# Autodesk Inventor assembly: Board Assembly
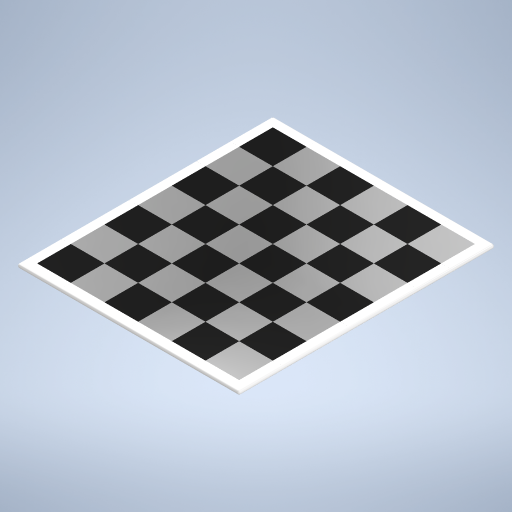
[picture p0: Inventor's stored thumbnail of the model, 512x512]
Saved by Autodesk Inventor 2023.1 (Build 271208000, 208)
## iProperties
Created: 2023-04-17
Part Number: Board Assembly
Document SubType Name: Assembly
Designer: czha626
Author: czha626
## Documents named in this file (9)
- C:\Users\czha626\OneDrive - The University of Auckland\Publications\Paper 2\Figures\Calibration target\Board Assembly.iam
- C:\Users\czha626\OneDrive - The University of Auckland\Publications\Paper 2\Calibration board\Calibration board\BoardNew2-CZ.ipt
- C:\Users\czha626\OneDrive - The University of Auckland\Publications\Paper 2\Calibration board\Calibration board\Connecter-CZ.ipt
- C:\Users\czha626\OneDrive - The University of Auckland\Publications\Paper 2\Calibration board\Calibration board\Boardborder.ipt
- C:\Users\czha626\OneDrive - The University of Auckland\Publications\Paper 2\Calibration board\Calibration board\Boardborder1.ipt
- C:\Users\czha626\OneDrive - The University of Auckland\Publications\Paper 2\Calibration board\Calibration board\Boardborder4.ipt
- C:\Users\czha626\OneDrive - The University of Auckland\Publications\Paper 2\Calibration board\Calibration board\Boardborder3.ipt
- C:\Users\czha626\OneDrive - The University of Auckland\Publications\Paper 2\Calibration board\Calibration board\Boardborder2.ipt
- C:\Users\czha626\OneDrive - The University of Auckland\Publications\Paper 2\Figures\Calibration target\Aluminium.ipt
## Components (132 placed, 8 different names)
1. BoardNew2-CZ:1 — Mate:1, Flush:1, Mate:2, Mate:3, Mate:4, Mate:5, Mate:7, Flush:2, Mate:29, Flush:9, Flush:10, Mate:31, Mate:32, Mate:34, Mate:52, Mate:53, Mate:54, Mate:198, Mate:199, Mate:209, Mate:259, Flush:46, Mate:326, Mate:328, Mate:329
2. Connecter-CZ:1 — Mate:19, Mate:20, Mate:21
3. Connecter-CZ:2 — Mate:16, Mate:17, Mate:18
4. Connecter-CZ:3 — Mate:2, Mate:3, Mate:4
5. Connecter-CZ:4 — Mate:5, Mate:6, Mate:7
6. BoardNew2-CZ:2 — Mate:1, Flush:1, Mate:6, Flush:2, Mate:15, Flush:5, Flush:6, Mate:16, Mate:21, Mate:49, Mate:50, Mate:51, Mate:196, Mate:197, Mate:210, Mate:311, Mate:320, Mate:325
7. BoardNew2-CZ:3 — Mate:15, Flush:5, Flush:6, Mate:17, Mate:18, Mate:19, Mate:20, Mate:46, Mate:47, Mate:48, Mate:194, Mate:195, Mate:211, Mate:257, Flush:45, Mate:319
8. Connecter-CZ:5
9. Connecter-CZ:6
10. BoardNew2-CZ:4 — Mate:43, Mate:44, Mate:45, Mate:127, Flush:25, Flush:26, Mate:192, Mate:193, Mate:212, Mate:213, Mate:214, Mate:215, Mate:216, Mate:217, Mate:230, Mate:255, Mate:256, Flush:44, Flush:54, Mate:322
11. BoardNew2-CZ:5 — Flush:11, Flush:12, Mate:36, Mate:37, Mate:39, Mate:40, Mate:42, Mate:58, Mate:59, Mate:60, Mate:202, Mate:203, Mate:207, Mate:265, Flush:49, Mate:332, Mate:334
12. Connecter-CZ:9
13. Connecter-CZ:10
14. BoardNew2-CZ:6 — Mate:29, Flush:9, Flush:10, Mate:30, Mate:33, Mate:35, Mate:55, Mate:56, Mate:57, Mate:200, Mate:201, Mate:208, Mate:330, Mate:331, Mate:333
15. Connecter-CZ:11 — Mate:192, Mate:193, Mate:212
16. Connecter-CZ:12 — Mate:30, Mate:31, Mate:32
17. Connecter-CZ:13 — Mate:33, Mate:34, Mate:35
18. BoardNew2-CZ:7 — Flush:11, Flush:12, Mate:36, Mate:38, Mate:41, Mate:61, Mate:62, Mate:63, Mate:204, Mate:205, Mate:206, Mate:231, Mate:232, Mate:233, Mate:234, Mate:243, Mate:244, Mate:249, Mate:250, Flush:41, Flush:51, Mate:302, Mate:335, Mate:337, Mate:339
19. Connecter-CZ:14 — Mate:40, Mate:41, Mate:42
20. Connecter-CZ:15 — Mate:37, Mate:38, Mate:39
21. Connecter-CZ:16 — Mate:43, Mate:44, Mate:45
22. Connecter-CZ:17 — Mate:49, Mate:50, Mate:51
23. Connecter-CZ:18 — Mate:52, Mate:53, Mate:54
24. Connecter-CZ:19 — Mate:46, Mate:47, Mate:48
25. Connecter-CZ:20 — Mate:55, Mate:56, Mate:57
26. Connecter-CZ:21 — Mate:58, Mate:59, Mate:60
27. Connecter-CZ:22 — Mate:61, Mate:62, Mate:63
28. BoardNew2-CZ:8 — Mate:305, Mate:307, Mate:312
29. Connecter-CZ:23
30. Connecter-CZ:24
31. Connecter-CZ:25
32. Connecter-CZ:26
33. BoardNew2-CZ:9 — Mate:285, Mate:310, Mate:315
34. BoardNew2-CZ:10 — Mate:313, Mate:314, Mate:317, Mate:321
35. Connecter-CZ:27
36. Connecter-CZ:28
37. BoardNew2-CZ:11 — Mate:127, Flush:25, Flush:26, Mate:191, Flush:39, Flush:40, Mate:218, Mate:219, Mate:220, Mate:221, Mate:228, Mate:229, Flush:53, Mate:275, Mate:282, Mate:316, Mate:318
38. BoardNew2-CZ:12 — Mate:298, Mate:336
39. Connecter-CZ:29
40. Connecter-CZ:30
41. BoardNew2-CZ:13 — Mate:291, Mate:300, Mate:304, Mate:306, Mate:309
42. Connecter-CZ:31
43. Connecter-CZ:32
44. BoardNew2-CZ:14 — Mate:235, Mate:236, Mate:237, Mate:238, Mate:245, Mate:246, Flush:52, Mate:301
45. Connecter-CZ:33
46. Connecter-CZ:34
47. Connecter-CZ:35
48. Connecter-CZ:36
49. Connecter-CZ:37
50. Connecter-CZ:38
51. Connecter-CZ:39
52. Connecter-CZ:40
53. Connecter-CZ:41
54. BoardNew2-CZ:15 — Mate:263, Flush:48, Mate:286, Mate:287, Mate:290, Mate:308
55. Connecter-CZ:42
56. Connecter-CZ:43
57. Connecter-CZ:44
58. Connecter-CZ:45
59. BoardNew2-CZ:16 — Mate:278, Mate:283
60. BoardNew2-CZ:17 — Mate:261, Flush:47, Mate:277, Mate:279, Mate:284
61. Connecter-CZ:46
62. Connecter-CZ:47
63. BoardNew2-CZ:18 — Mate:191, Flush:39, Flush:40, Mate:222, Mate:223, Mate:224, Mate:225, Mate:226, Mate:227, Mate:251, Mate:252, Flush:42, Mate:273, Mate:280
64. BoardNew2-CZ:19 — Mate:267, Flush:50, Mate:292, Mate:296, Mate:299
65. Connecter-CZ:48
66. Connecter-CZ:49
67. BoardNew2-CZ:20 — Mate:288, Mate:289, Mate:293
68. Connecter-CZ:50
69. Connecter-CZ:51
70. BoardNew2-CZ:21 — Mate:239, Mate:240, Mate:241, Mate:242, Mate:247, Mate:248, Mate:253, Mate:254, Flush:43, Mate:269, Mate:271, Mate:295, Mate:297
71. Connecter-CZ:52
72. Connecter-CZ:53
73. Connecter-CZ:54
74. Connecter-CZ:55
75. Connecter-CZ:56
76. Connecter-CZ:57
77. Connecter-CZ:58
78. Connecter-CZ:59
79. Connecter-CZ:60
80. Connecter-CZ:61 — Mate:198, Mate:199, Mate:209
81. Connecter-CZ:62 — Mate:200, Mate:201, Mate:208
82. Connecter-CZ:63 — Mate:194, Mate:195, Mate:211
83. Connecter-CZ:64 — Mate:202, Mate:203, Mate:207
84. Connecter-CZ:65 — Mate:204, Mate:205, Mate:206
85. Connecter-CZ:66 — Mate:196, Mate:197, Mate:210
86. Connecter-CZ:67 — Mate:213, Mate:214, Mate:215
87. Connecter-CZ:68 — Mate:216, Mate:217, Mate:230
88. Connecter-CZ:69 — Mate:218, Mate:219, Mate:229
89. Connecter-CZ:70 — Mate:220, Mate:221, Mate:228
90. Connecter-CZ:71 — Mate:222, Mate:223, Mate:227
91. Connecter-CZ:72 — Mate:224, Mate:225, Mate:226
92. Connecter-CZ:73 — Mate:231, Mate:232, Mate:243
93. Connecter-CZ:74 — Mate:233, Mate:234, Mate:244
94. Connecter-CZ:75 — Mate:235, Mate:236, Mate:245
95. Connecter-CZ:76 — Mate:237, Mate:238, Mate:246
96. Connecter-CZ:77 — Mate:239, Mate:240, Mate:247
97. Connecter-CZ:78 — Mate:241, Mate:242, Mate:248
98. Boardborder:1 — Mate:249, Mate:250, Flush:41, Mate:270, Mate:338
99. Boardborder:2 — Mate:251, Mate:252, Flush:42, Mate:262, Mate:274
100. Boardborder1:1 — Mate:253, Mate:254, Flush:43, Mate:268
101. Boardborder1:2 — Mate:255, Mate:256, Flush:44, Mate:258, Mate:276, Mate:323, Mate:324
102. Boardborder4:1 — Mate:257, Mate:258, Flush:45, Mate:260, Mate:327
103. Boardborder4:2 — Mate:261, Flush:47, Mate:262, Mate:264
104. Boardborder4:3 — Mate:259, Flush:46, Mate:260, Mate:266
105. Boardborder4:4 — Mate:263, Flush:48, Mate:264
106. Boardborder3:1 — Mate:267, Mate:268, Flush:50, Mate:294
107. Boardborder3:2 — Mate:265, Flush:49, Mate:266
108. Boardborder2:1 — Mate:269, Mate:270, Flush:51, Mate:272, Mate:303
109. Boardborder2:2 — Mate:271, Mate:272, Flush:52
110. Boardborder2:3 — Mate:275, Mate:276, Flush:54
111. Boardborder2:4 — Mate:273, Mate:274, Flush:53, Mate:281
112. Aluminium:1 — Mate:277, Mate:278, Mate:279
113. Aluminium:2 — Mate:283, Mate:284, Mate:285
114. Aluminium:3 — Mate:280, Mate:281, Mate:282
115. Aluminium:4 — Mate:286, Mate:287, Mate:288
116. Aluminium:5 — Mate:289, Mate:290, Mate:291
117. Aluminium:6 — Mate:292, Mate:293, Mate:294
118. Aluminium:7 — Mate:301, Mate:302, Mate:303
119. Aluminium:8 — Mate:298, Mate:299, Mate:300
120. Aluminium:9 — Mate:295, Mate:296, Mate:297
121. Aluminium:10 — Mate:322, Mate:323, Mate:324
122. Aluminium:11 — Mate:319, Mate:320, Mate:321
123. Aluminium:12 — Mate:310, Mate:311, Mate:312
124. Aluminium:13 — Mate:313, Mate:314, Mate:315
125. Aluminium:14 — Mate:307, Mate:308, Mate:309
126. Aluminium:15 — Mate:304, Mate:305, Mate:306
127. Aluminium:16 — Mate:316, Mate:317, Mate:318
128. Aluminium:17 — Mate:325, Mate:326, Mate:327
129. Aluminium:18 — Mate:337, Mate:338, Mate:339
130. Aluminium:19 — Mate:334, Mate:335, Mate:336
131. Aluminium:20 — Mate:331, Mate:332, Mate:333
132. Aluminium:21 — Mate:328, Mate:329, Mate:330
## Relationships (393: Mate 339, Flush 54)
- Mate:1: BoardNew2-CZ:1 ↔ BoardNew2-CZ:2
- Flush:1: BoardNew2-CZ:1 ↔ BoardNew2-CZ:2
- Mate:2: BoardNew2-CZ:1 ↔ Connecter-CZ:3
- Mate:3: BoardNew2-CZ:1 ↔ Connecter-CZ:3
- Mate:4: BoardNew2-CZ:1 ↔ Connecter-CZ:3
- Mate:5: BoardNew2-CZ:1 ↔ Connecter-CZ:4
- Mate:6: Connecter-CZ:4 ↔ BoardNew2-CZ:2
- Mate:7: BoardNew2-CZ:1 ↔ Connecter-CZ:4
- Flush:2: BoardNew2-CZ:1 ↔ BoardNew2-CZ:2
- [Mate]: BoardNew2-CZ:3 ↔ BoardNew2-CZ:4
- [Flush]: BoardNew2-CZ:3 ↔ BoardNew2-CZ:4
- [Mate]: BoardNew2-CZ:3 ↔ Connecter-CZ:5
- [Mate]: BoardNew2-CZ:3 ↔ Connecter-CZ:5
- [Mate]: BoardNew2-CZ:3 ↔ Connecter-CZ:5
- [Mate]: BoardNew2-CZ:3 ↔ Connecter-CZ:6
- [Mate]: Connecter-CZ:6 ↔ BoardNew2-CZ:4
- [Mate]: BoardNew2-CZ:3 ↔ Connecter-CZ:6
- [Flush]: BoardNew2-CZ:3 ↔ BoardNew2-CZ:4
- Mate:15: BoardNew2-CZ:2 ↔ BoardNew2-CZ:3
- Flush:5: BoardNew2-CZ:2 ↔ BoardNew2-CZ:3
- Flush:6: BoardNew2-CZ:2 ↔ BoardNew2-CZ:3
- Mate:16: Connecter-CZ:2 ↔ BoardNew2-CZ:2
- Mate:17: Connecter-CZ:2 ↔ BoardNew2-CZ:3
- Mate:18: Connecter-CZ:2 ↔ BoardNew2-CZ:3
- Mate:19: Connecter-CZ:1 ↔ BoardNew2-CZ:3
- Mate:20: Connecter-CZ:1 ↔ BoardNew2-CZ:3
- Mate:21: Connecter-CZ:1 ↔ BoardNew2-CZ:2
- [Mate]: BoardNew2-CZ:5 ↔ BoardNew2-CZ:6
- [Flush]: BoardNew2-CZ:5 ↔ BoardNew2-CZ:6
- [Mate]: BoardNew2-CZ:5 ↔ Connecter-CZ:9
- [Mate]: BoardNew2-CZ:5 ↔ Connecter-CZ:9
- [Mate]: BoardNew2-CZ:5 ↔ Connecter-CZ:9
- [Mate]: BoardNew2-CZ:5 ↔ Connecter-CZ:10
- [Mate]: Connecter-CZ:10 ↔ BoardNew2-CZ:6
- [Mate]: BoardNew2-CZ:5 ↔ Connecter-CZ:10
- [Flush]: BoardNew2-CZ:5 ↔ BoardNew2-CZ:6
- Mate:29: BoardNew2-CZ:1 ↔ BoardNew2-CZ:6
- Flush:9: BoardNew2-CZ:1 ↔ BoardNew2-CZ:6
- Flush:10: BoardNew2-CZ:1 ↔ BoardNew2-CZ:6
- Mate:30: BoardNew2-CZ:6 ↔ Connecter-CZ:12
- Mate:31: BoardNew2-CZ:1 ↔ Connecter-CZ:12
- Mate:32: BoardNew2-CZ:1 ↔ Connecter-CZ:12
- Mate:33: BoardNew2-CZ:6 ↔ Connecter-CZ:13
- Mate:34: BoardNew2-CZ:1 ↔ Connecter-CZ:13
- Mate:35: BoardNew2-CZ:6 ↔ Connecter-CZ:13
- Flush:11: BoardNew2-CZ:5 ↔ BoardNew2-CZ:7
- Flush:12: BoardNew2-CZ:5 ↔ BoardNew2-CZ:7
- Mate:36: BoardNew2-CZ:5 ↔ BoardNew2-CZ:7
- Mate:37: BoardNew2-CZ:5 ↔ Connecter-CZ:15
- Mate:38: BoardNew2-CZ:7 ↔ Connecter-CZ:15
- Mate:39: BoardNew2-CZ:5 ↔ Connecter-CZ:15
- Mate:40: BoardNew2-CZ:5 ↔ Connecter-CZ:14
- Mate:41: BoardNew2-CZ:7 ↔ Connecter-CZ:14
- Mate:42: BoardNew2-CZ:5 ↔ Connecter-CZ:14
- Mate:43: BoardNew2-CZ:4 ↔ Connecter-CZ:16
- Mate:44: BoardNew2-CZ:4 ↔ Connecter-CZ:16
- Mate:45: BoardNew2-CZ:4 ↔ Connecter-CZ:16
- Mate:46: BoardNew2-CZ:3 ↔ Connecter-CZ:19
- Mate:47: BoardNew2-CZ:3 ↔ Connecter-CZ:19
- Mate:48: BoardNew2-CZ:3 ↔ Connecter-CZ:19
- Mate:49: BoardNew2-CZ:2 ↔ Connecter-CZ:17
- Mate:50: BoardNew2-CZ:2 ↔ Connecter-CZ:17
- Mate:51: BoardNew2-CZ:2 ↔ Connecter-CZ:17
- Mate:52: BoardNew2-CZ:1 ↔ Connecter-CZ:18
- Mate:53: BoardNew2-CZ:1 ↔ Connecter-CZ:18
- Mate:54: BoardNew2-CZ:1 ↔ Connecter-CZ:18
- Mate:55: BoardNew2-CZ:6 ↔ Connecter-CZ:20
- Mate:56: BoardNew2-CZ:6 ↔ Connecter-CZ:20
- Mate:57: BoardNew2-CZ:6 ↔ Connecter-CZ:20
- Mate:58: BoardNew2-CZ:5 ↔ Connecter-CZ:21
- Mate:59: BoardNew2-CZ:5 ↔ Connecter-CZ:21
- Mate:60: BoardNew2-CZ:5 ↔ Connecter-CZ:21
- Mate:61: BoardNew2-CZ:7 ↔ Connecter-CZ:22
- Mate:62: BoardNew2-CZ:7 ↔ Connecter-CZ:22
- Mate:63: BoardNew2-CZ:7 ↔ Connecter-CZ:22
- [Mate]: BoardNew2-CZ:8 ↔ BoardNew2-CZ:9
- [Flush]: BoardNew2-CZ:8 ↔ BoardNew2-CZ:9
- [Mate]: BoardNew2-CZ:8 ↔ Connecter-CZ:25
- [Mate]: BoardNew2-CZ:8 ↔ Connecter-CZ:25
- [Mate]: BoardNew2-CZ:8 ↔ Connecter-CZ:25
- [Mate]: BoardNew2-CZ:8 ↔ Connecter-CZ:26
- [Mate]: Connecter-CZ:26 ↔ BoardNew2-CZ:9
- [Mate]: BoardNew2-CZ:8 ↔ Connecter-CZ:26
- [Flush]: BoardNew2-CZ:8 ↔ BoardNew2-CZ:9
- [Mate]: BoardNew2-CZ:10 ↔ BoardNew2-CZ:11
- [Flush]: BoardNew2-CZ:10 ↔ BoardNew2-CZ:11
- [Mate]: BoardNew2-CZ:10 ↔ Connecter-CZ:27
- [Mate]: BoardNew2-CZ:10 ↔ Connecter-CZ:27
- [Mate]: BoardNew2-CZ:10 ↔ Connecter-CZ:27
- [Mate]: BoardNew2-CZ:10 ↔ Connecter-CZ:28
- [Mate]: Connecter-CZ:28 ↔ BoardNew2-CZ:11
- [Mate]: BoardNew2-CZ:10 ↔ Connecter-CZ:28
- [Flush]: BoardNew2-CZ:10 ↔ BoardNew2-CZ:11
- [Mate]: BoardNew2-CZ:9 ↔ BoardNew2-CZ:10
- [Flush]: BoardNew2-CZ:9 ↔ BoardNew2-CZ:10
- [Flush]: BoardNew2-CZ:9 ↔ BoardNew2-CZ:10
- [Mate]: Connecter-CZ:24 ↔ BoardNew2-CZ:9
- [Mate]: Connecter-CZ:24 ↔ BoardNew2-CZ:10
- [Mate]: Connecter-CZ:24 ↔ BoardNew2-CZ:10
- [Mate]: Connecter-CZ:23 ↔ BoardNew2-CZ:10
- [Mate]: Connecter-CZ:23 ↔ BoardNew2-CZ:10
- [Mate]: Connecter-CZ:23 ↔ BoardNew2-CZ:9
- [Mate]: BoardNew2-CZ:12 ↔ BoardNew2-CZ:13
- [Flush]: BoardNew2-CZ:12 ↔ BoardNew2-CZ:13
- [Mate]: BoardNew2-CZ:12 ↔ Connecter-CZ:29
- [Mate]: BoardNew2-CZ:12 ↔ Connecter-CZ:29
- [Mate]: BoardNew2-CZ:12 ↔ Connecter-CZ:29
- [Mate]: BoardNew2-CZ:12 ↔ Connecter-CZ:30
- [Mate]: Connecter-CZ:30 ↔ BoardNew2-CZ:13
- [Mate]: BoardNew2-CZ:12 ↔ Connecter-CZ:30
- [Flush]: BoardNew2-CZ:12 ↔ BoardNew2-CZ:13
- [Mate]: BoardNew2-CZ:8 ↔ BoardNew2-CZ:13
- [Flush]: BoardNew2-CZ:8 ↔ BoardNew2-CZ:13
- [Flush]: BoardNew2-CZ:8 ↔ BoardNew2-CZ:13
- [Mate]: BoardNew2-CZ:13 ↔ Connecter-CZ:31
- [Mate]: BoardNew2-CZ:8 ↔ Connecter-CZ:31
- [Mate]: BoardNew2-CZ:8 ↔ Connecter-CZ:31
- [Mate]: BoardNew2-CZ:13 ↔ Connecter-CZ:32
- [Mate]: BoardNew2-CZ:8 ↔ Connecter-CZ:32
- [Mate]: BoardNew2-CZ:13 ↔ Connecter-CZ:32
- [Flush]: BoardNew2-CZ:12 ↔ BoardNew2-CZ:14
- [Flush]: BoardNew2-CZ:12 ↔ BoardNew2-CZ:14
- [Mate]: BoardNew2-CZ:12 ↔ BoardNew2-CZ:14
- [Mate]: BoardNew2-CZ:12 ↔ Connecter-CZ:34
- [Mate]: BoardNew2-CZ:14 ↔ Connecter-CZ:34
- [Mate]: BoardNew2-CZ:12 ↔ Connecter-CZ:34
- [Mate]: BoardNew2-CZ:12 ↔ Connecter-CZ:33
- [Mate]: BoardNew2-CZ:14 ↔ Connecter-CZ:33
- [Mate]: BoardNew2-CZ:12 ↔ Connecter-CZ:33
- [Mate]: BoardNew2-CZ:11 ↔ Connecter-CZ:35
- [Mate]: BoardNew2-CZ:11 ↔ Connecter-CZ:35
- [Mate]: BoardNew2-CZ:11 ↔ Connecter-CZ:35
- [Mate]: BoardNew2-CZ:10 ↔ Connecter-CZ:38
- [Mate]: BoardNew2-CZ:10 ↔ Connecter-CZ:38
- [Mate]: BoardNew2-CZ:10 ↔ Connecter-CZ:38
- [Mate]: BoardNew2-CZ:9 ↔ Connecter-CZ:36
- [Mate]: BoardNew2-CZ:9 ↔ Connecter-CZ:36
- [Mate]: BoardNew2-CZ:9 ↔ Connecter-CZ:36
- [Mate]: BoardNew2-CZ:8 ↔ Connecter-CZ:37
- [Mate]: BoardNew2-CZ:8 ↔ Connecter-CZ:37
- [Mate]: BoardNew2-CZ:8 ↔ Connecter-CZ:37
- [Mate]: BoardNew2-CZ:13 ↔ Connecter-CZ:39
- [Mate]: BoardNew2-CZ:13 ↔ Connecter-CZ:39
- [Mate]: BoardNew2-CZ:13 ↔ Connecter-CZ:39
- [Mate]: BoardNew2-CZ:12 ↔ Connecter-CZ:40
- [Mate]: BoardNew2-CZ:12 ↔ Connecter-CZ:40
- [Mate]: BoardNew2-CZ:12 ↔ Connecter-CZ:40
- [Mate]: BoardNew2-CZ:14 ↔ Connecter-CZ:41
- [Mate]: BoardNew2-CZ:14 ↔ Connecter-CZ:41
- [Mate]: BoardNew2-CZ:14 ↔ Connecter-CZ:41
- Mate:127: BoardNew2-CZ:4 ↔ BoardNew2-CZ:11
- Flush:25: BoardNew2-CZ:4 ↔ BoardNew2-CZ:11
- Flush:26: BoardNew2-CZ:4 ↔ BoardNew2-CZ:11
- [Mate]: BoardNew2-CZ:15 ↔ BoardNew2-CZ:16
- [Flush]: BoardNew2-CZ:15 ↔ BoardNew2-CZ:16
- [Mate]: BoardNew2-CZ:15 ↔ Connecter-CZ:44
- [Mate]: BoardNew2-CZ:15 ↔ Connecter-CZ:44
- [Mate]: BoardNew2-CZ:15 ↔ Connecter-CZ:44
- [Mate]: BoardNew2-CZ:15 ↔ Connecter-CZ:45
- [Mate]: Connecter-CZ:45 ↔ BoardNew2-CZ:16
- [Mate]: BoardNew2-CZ:15 ↔ Connecter-CZ:45
- [Flush]: BoardNew2-CZ:15 ↔ BoardNew2-CZ:16
- [Mate]: BoardNew2-CZ:17 ↔ BoardNew2-CZ:18
- [Flush]: BoardNew2-CZ:17 ↔ BoardNew2-CZ:18
- [Mate]: BoardNew2-CZ:17 ↔ Connecter-CZ:46
- [Mate]: BoardNew2-CZ:17 ↔ Connecter-CZ:46
- [Mate]: BoardNew2-CZ:17 ↔ Connecter-CZ:46
- [Mate]: BoardNew2-CZ:17 ↔ Connecter-CZ:47
- [Mate]: Connecter-CZ:47 ↔ BoardNew2-CZ:18
- [Mate]: BoardNew2-CZ:17 ↔ Connecter-CZ:47
- [Flush]: BoardNew2-CZ:17 ↔ BoardNew2-CZ:18
- [Mate]: BoardNew2-CZ:16 ↔ BoardNew2-CZ:17
- [Flush]: BoardNew2-CZ:16 ↔ BoardNew2-CZ:17
- [Flush]: BoardNew2-CZ:16 ↔ BoardNew2-CZ:17
- [Mate]: Connecter-CZ:43 ↔ BoardNew2-CZ:16
- [Mate]: Connecter-CZ:43 ↔ BoardNew2-CZ:17
- [Mate]: Connecter-CZ:43 ↔ BoardNew2-CZ:17
- [Mate]: Connecter-CZ:42 ↔ BoardNew2-CZ:17
- [Mate]: Connecter-CZ:42 ↔ BoardNew2-CZ:17
- [Mate]: Connecter-CZ:42 ↔ BoardNew2-CZ:16
- [Mate]: BoardNew2-CZ:19 ↔ BoardNew2-CZ:20
- [Flush]: BoardNew2-CZ:19 ↔ BoardNew2-CZ:20
- [Mate]: BoardNew2-CZ:19 ↔ Connecter-CZ:48
- [Mate]: BoardNew2-CZ:19 ↔ Connecter-CZ:48
- [Mate]: BoardNew2-CZ:19 ↔ Connecter-CZ:48
- [Mate]: BoardNew2-CZ:19 ↔ Connecter-CZ:49
- [Mate]: Connecter-CZ:49 ↔ BoardNew2-CZ:20
- [Mate]: BoardNew2-CZ:19 ↔ Connecter-CZ:49
- [Flush]: BoardNew2-CZ:19 ↔ BoardNew2-CZ:20
- [Mate]: BoardNew2-CZ:15 ↔ BoardNew2-CZ:20
- [Flush]: BoardNew2-CZ:15 ↔ BoardNew2-CZ:20
- [Flush]: BoardNew2-CZ:15 ↔ BoardNew2-CZ:20
- [Mate]: BoardNew2-CZ:20 ↔ Connecter-CZ:50
- [Mate]: BoardNew2-CZ:15 ↔ Connecter-CZ:50
- [Mate]: BoardNew2-CZ:15 ↔ Connecter-CZ:50
- [Mate]: BoardNew2-CZ:20 ↔ Connecter-CZ:51
- [Mate]: BoardNew2-CZ:15 ↔ Connecter-CZ:51
- [Mate]: BoardNew2-CZ:20 ↔ Connecter-CZ:51
- [Flush]: BoardNew2-CZ:19 ↔ BoardNew2-CZ:21
- [Flush]: BoardNew2-CZ:19 ↔ BoardNew2-CZ:21
- [Mate]: BoardNew2-CZ:19 ↔ BoardNew2-CZ:21
- [Mate]: BoardNew2-CZ:19 ↔ Connecter-CZ:53
- [Mate]: BoardNew2-CZ:21 ↔ Connecter-CZ:53
- [Mate]: BoardNew2-CZ:19 ↔ Connecter-CZ:53
- [Mate]: BoardNew2-CZ:19 ↔ Connecter-CZ:52
- [Mate]: BoardNew2-CZ:21 ↔ Connecter-CZ:52
- [Mate]: BoardNew2-CZ:19 ↔ Connecter-CZ:52
- [Mate]: BoardNew2-CZ:18 ↔ Connecter-CZ:54
- [Mate]: BoardNew2-CZ:18 ↔ Connecter-CZ:54
- [Mate]: BoardNew2-CZ:18 ↔ Connecter-CZ:54
- [Mate]: BoardNew2-CZ:17 ↔ Connecter-CZ:57
- [Mate]: BoardNew2-CZ:17 ↔ Connecter-CZ:57
- [Mate]: BoardNew2-CZ:17 ↔ Connecter-CZ:57
- [Mate]: BoardNew2-CZ:16 ↔ Connecter-CZ:55
- [Mate]: BoardNew2-CZ:16 ↔ Connecter-CZ:55
- [Mate]: BoardNew2-CZ:16 ↔ Connecter-CZ:55
- [Mate]: BoardNew2-CZ:15 ↔ Connecter-CZ:56
- [Mate]: BoardNew2-CZ:15 ↔ Connecter-CZ:56
- [Mate]: BoardNew2-CZ:15 ↔ Connecter-CZ:56
- [Mate]: BoardNew2-CZ:20 ↔ Connecter-CZ:58
- [Mate]: BoardNew2-CZ:20 ↔ Connecter-CZ:58
- [Mate]: BoardNew2-CZ:20 ↔ Connecter-CZ:58
- [Mate]: BoardNew2-CZ:19 ↔ Connecter-CZ:59
- [Mate]: BoardNew2-CZ:19 ↔ Connecter-CZ:59
- [Mate]: BoardNew2-CZ:19 ↔ Connecter-CZ:59
- [Mate]: BoardNew2-CZ:21 ↔ Connecter-CZ:60
- [Mate]: BoardNew2-CZ:21 ↔ Connecter-CZ:60
- [Mate]: BoardNew2-CZ:21 ↔ Connecter-CZ:60
- Mate:191: BoardNew2-CZ:11 ↔ BoardNew2-CZ:18
- Flush:39: BoardNew2-CZ:11 ↔ BoardNew2-CZ:18
- Flush:40: BoardNew2-CZ:11 ↔ BoardNew2-CZ:18
- Mate:192: BoardNew2-CZ:4 ↔ Connecter-CZ:11
- Mate:193: BoardNew2-CZ:4 ↔ Connecter-CZ:11
- Mate:194: BoardNew2-CZ:3 ↔ Connecter-CZ:63
- Mate:195: BoardNew2-CZ:3 ↔ Connecter-CZ:63
- Mate:196: BoardNew2-CZ:2 ↔ Connecter-CZ:66
- Mate:197: BoardNew2-CZ:2 ↔ Connecter-CZ:66
- Mate:198: BoardNew2-CZ:1 ↔ Connecter-CZ:61
- Mate:199: BoardNew2-CZ:1 ↔ Connecter-CZ:61
- Mate:200: BoardNew2-CZ:6 ↔ Connecter-CZ:62
- Mate:201: BoardNew2-CZ:6 ↔ Connecter-CZ:62
- Mate:202: BoardNew2-CZ:5 ↔ Connecter-CZ:64
- Mate:203: BoardNew2-CZ:5 ↔ Connecter-CZ:64
- Mate:204: BoardNew2-CZ:7 ↔ Connecter-CZ:65
- Mate:205: BoardNew2-CZ:7 ↔ Connecter-CZ:65
- Mate:206: BoardNew2-CZ:7 ↔ Connecter-CZ:65
- Mate:207: BoardNew2-CZ:5 ↔ Connecter-CZ:64
- Mate:208: BoardNew2-CZ:6 ↔ Connecter-CZ:62
- Mate:209: BoardNew2-CZ:1 ↔ Connecter-CZ:61
- Mate:210: BoardNew2-CZ:2 ↔ Connecter-CZ:66
- Mate:211: BoardNew2-CZ:3 ↔ Connecter-CZ:63
- Mate:212: BoardNew2-CZ:4 ↔ Connecter-CZ:11
- Mate:213: BoardNew2-CZ:4 ↔ Connecter-CZ:67
- Mate:214: BoardNew2-CZ:4 ↔ Connecter-CZ:67
- Mate:215: BoardNew2-CZ:4 ↔ Connecter-CZ:67
- Mate:216: BoardNew2-CZ:4 ↔ Connecter-CZ:68
- Mate:217: BoardNew2-CZ:4 ↔ Connecter-CZ:68
- Mate:218: BoardNew2-CZ:11 ↔ Connecter-CZ:69
- Mate:219: BoardNew2-CZ:11 ↔ Connecter-CZ:69
- Mate:220: BoardNew2-CZ:11 ↔ Connecter-CZ:70
- Mate:221: BoardNew2-CZ:11 ↔ Connecter-CZ:70
- Mate:222: BoardNew2-CZ:18 ↔ Connecter-CZ:71
- Mate:223: BoardNew2-CZ:18 ↔ Connecter-CZ:71
- Mate:224: BoardNew2-CZ:18 ↔ Connecter-CZ:72
- Mate:225: BoardNew2-CZ:18 ↔ Connecter-CZ:72
- Mate:226: BoardNew2-CZ:18 ↔ Connecter-CZ:72
- Mate:227: BoardNew2-CZ:18 ↔ Connecter-CZ:71
- Mate:228: BoardNew2-CZ:11 ↔ Connecter-CZ:70
- Mate:229: BoardNew2-CZ:11 ↔ Connecter-CZ:69
- Mate:230: BoardNew2-CZ:4 ↔ Connecter-CZ:68
- Mate:231: BoardNew2-CZ:7 ↔ Connecter-CZ:73
- Mate:232: BoardNew2-CZ:7 ↔ Connecter-CZ:73
- Mate:233: BoardNew2-CZ:7 ↔ Connecter-CZ:74
- Mate:234: BoardNew2-CZ:7 ↔ Connecter-CZ:74
- Mate:235: BoardNew2-CZ:14 ↔ Connecter-CZ:75
- Mate:236: BoardNew2-CZ:14 ↔ Connecter-CZ:75
- Mate:237: BoardNew2-CZ:14 ↔ Connecter-CZ:76
- Mate:238: BoardNew2-CZ:14 ↔ Connecter-CZ:76
- Mate:239: BoardNew2-CZ:21 ↔ Connecter-CZ:77
- Mate:240: BoardNew2-CZ:21 ↔ Connecter-CZ:77
- Mate:241: BoardNew2-CZ:21 ↔ Connecter-CZ:78
- Mate:242: BoardNew2-CZ:21 ↔ Connecter-CZ:78
- Mate:243: BoardNew2-CZ:7 ↔ Connecter-CZ:73
- Mate:244: BoardNew2-CZ:7 ↔ Connecter-CZ:74
- Mate:245: BoardNew2-CZ:14 ↔ Connecter-CZ:75
- Mate:246: BoardNew2-CZ:14 ↔ Connecter-CZ:76
- Mate:247: BoardNew2-CZ:21 ↔ Connecter-CZ:77
- Mate:248: BoardNew2-CZ:21 ↔ Connecter-CZ:78
- Mate:249: BoardNew2-CZ:7 ↔ Boardborder:1
- Mate:250: BoardNew2-CZ:7 ↔ Boardborder:1
- Flush:41: BoardNew2-CZ:7 ↔ Boardborder:1
- Mate:251: BoardNew2-CZ:18 ↔ Boardborder:2
- Mate:252: BoardNew2-CZ:18 ↔ Boardborder:2
- Flush:42: BoardNew2-CZ:18 ↔ Boardborder:2
- Mate:253: BoardNew2-CZ:21 ↔ Boardborder1:1
- Mate:254: BoardNew2-CZ:21 ↔ Boardborder1:1
- Flush:43: BoardNew2-CZ:21 ↔ Boardborder1:1
- Mate:255: BoardNew2-CZ:4 ↔ Boardborder1:2
- Mate:256: BoardNew2-CZ:4 ↔ Boardborder1:2
- Flush:44: BoardNew2-CZ:4 ↔ Boardborder1:2
- Mate:257: BoardNew2-CZ:3 ↔ Boardborder4:1
- Mate:258: Boardborder1:2 ↔ Boardborder4:1
- Flush:45: BoardNew2-CZ:3 ↔ Boardborder4:1
- Mate:259: BoardNew2-CZ:1 ↔ Boardborder4:3
- Flush:46: BoardNew2-CZ:1 ↔ Boardborder4:3
- Mate:260: Boardborder4:1 ↔ Boardborder4:3
- Mate:261: BoardNew2-CZ:17 ↔ Boardborder4:2
- Flush:47: BoardNew2-CZ:17 ↔ Boardborder4:2
- Mate:262: Boardborder:2 ↔ Boardborder4:2
- Mate:263: BoardNew2-CZ:15 ↔ Boardborder4:4
- Flush:48: BoardNew2-CZ:15 ↔ Boardborder4:4
- Mate:264: Boardborder4:2 ↔ Boardborder4:4
- Mate:265: BoardNew2-CZ:5 ↔ Boardborder3:2
- Flush:49: BoardNew2-CZ:5 ↔ Boardborder3:2
- Mate:266: Boardborder4:3 ↔ Boardborder3:2
- Mate:267: BoardNew2-CZ:19 ↔ Boardborder3:1
- Mate:268: Boardborder1:1 ↔ Boardborder3:1
- Flush:50: BoardNew2-CZ:19 ↔ Boardborder3:1
- Mate:269: BoardNew2-CZ:21 ↔ Boardborder2:1
- Mate:270: Boardborder:1 ↔ Boardborder2:1
- Flush:51: BoardNew2-CZ:7 ↔ Boardborder2:1
- Mate:271: BoardNew2-CZ:21 ↔ Boardborder2:2
- Mate:272: Boardborder2:1 ↔ Boardborder2:2
- Flush:52: BoardNew2-CZ:14 ↔ Boardborder2:2
- Mate:273: BoardNew2-CZ:18 ↔ Boardborder2:4
- Mate:274: Boardborder:2 ↔ Boardborder2:4
- Flush:53: BoardNew2-CZ:11 ↔ Boardborder2:4
- Mate:275: BoardNew2-CZ:11 ↔ Boardborder2:3
- Mate:276: Boardborder1:2 ↔ Boardborder2:3
- Flush:54: BoardNew2-CZ:4 ↔ Boardborder2:3
- Mate:277: BoardNew2-CZ:17 ↔ Aluminium:1
- Mate:278: BoardNew2-CZ:16 ↔ Aluminium:1
- Mate:279: BoardNew2-CZ:17 ↔ Aluminium:1
- Mate:280: BoardNew2-CZ:18 ↔ Aluminium:3
- Mate:281: Boardborder2:4 ↔ Aluminium:3
- Mate:282: BoardNew2-CZ:11 ↔ Aluminium:3
- Mate:283: BoardNew2-CZ:16 ↔ Aluminium:2
- Mate:284: BoardNew2-CZ:17 ↔ Aluminium:2
- Mate:285: BoardNew2-CZ:9 ↔ Aluminium:2
- Mate:286: BoardNew2-CZ:15 ↔ Aluminium:4
- Mate:287: BoardNew2-CZ:15 ↔ Aluminium:4
- Mate:288: BoardNew2-CZ:20 ↔ Aluminium:4
- Mate:289: BoardNew2-CZ:20 ↔ Aluminium:5
- Mate:290: BoardNew2-CZ:15 ↔ Aluminium:5
- Mate:291: BoardNew2-CZ:13 ↔ Aluminium:5
- Mate:292: BoardNew2-CZ:19 ↔ Aluminium:6
- Mate:293: BoardNew2-CZ:20 ↔ Aluminium:6
- Mate:294: Boardborder3:1 ↔ Aluminium:6
- Mate:295: BoardNew2-CZ:21 ↔ Aluminium:9
- Mate:296: BoardNew2-CZ:19 ↔ Aluminium:9
- Mate:297: BoardNew2-CZ:21 ↔ Aluminium:9
- Mate:298: BoardNew2-CZ:12 ↔ Aluminium:8
- Mate:299: BoardNew2-CZ:19 ↔ Aluminium:8
- Mate:300: BoardNew2-CZ:13 ↔ Aluminium:8
- Mate:301: BoardNew2-CZ:14 ↔ Aluminium:7
- Mate:302: BoardNew2-CZ:7 ↔ Aluminium:7
- Mate:303: Boardborder2:1 ↔ Aluminium:7
- Mate:304: BoardNew2-CZ:13 ↔ Aluminium:15
- Mate:305: BoardNew2-CZ:8 ↔ Aluminium:15
- Mate:306: BoardNew2-CZ:13 ↔ Aluminium:15
- Mate:307: BoardNew2-CZ:8 ↔ Aluminium:14
- Mate:308: BoardNew2-CZ:15 ↔ Aluminium:14
- Mate:309: BoardNew2-CZ:13 ↔ Aluminium:14
- Mate:310: BoardNew2-CZ:9 ↔ Aluminium:12
- Mate:311: BoardNew2-CZ:2 ↔ Aluminium:12
- Mate:312: BoardNew2-CZ:8 ↔ Aluminium:12
- Mate:313: BoardNew2-CZ:10 ↔ Aluminium:13
- Mate:314: BoardNew2-CZ:10 ↔ Aluminium:13
- Mate:315: BoardNew2-CZ:9 ↔ Aluminium:13
- Mate:316: BoardNew2-CZ:11 ↔ Aluminium:16
- Mate:317: BoardNew2-CZ:10 ↔ Aluminium:16
- Mate:318: BoardNew2-CZ:11 ↔ Aluminium:16
- Mate:319: BoardNew2-CZ:3 ↔ Aluminium:11
- Mate:320: BoardNew2-CZ:2 ↔ Aluminium:11
- Mate:321: BoardNew2-CZ:10 ↔ Aluminium:11
- Mate:322: BoardNew2-CZ:4 ↔ Aluminium:10
- Mate:323: Boardborder1:2 ↔ Aluminium:10
- Mate:324: Boardborder1:2 ↔ Aluminium:10
- Mate:325: BoardNew2-CZ:2 ↔ Aluminium:17
- Mate:326: BoardNew2-CZ:1 ↔ Aluminium:17
- Mate:327: Boardborder4:1 ↔ Aluminium:17
- Mate:328: BoardNew2-CZ:1 ↔ Aluminium:21
- Mate:329: BoardNew2-CZ:1 ↔ Aluminium:21
- Mate:330: BoardNew2-CZ:6 ↔ Aluminium:21
- Mate:331: BoardNew2-CZ:6 ↔ Aluminium:20
- Mate:332: BoardNew2-CZ:5 ↔ Aluminium:20
- Mate:333: BoardNew2-CZ:6 ↔ Aluminium:20
- Mate:334: BoardNew2-CZ:5 ↔ Aluminium:19
- Mate:335: BoardNew2-CZ:7 ↔ Aluminium:19
- Mate:336: BoardNew2-CZ:12 ↔ Aluminium:19
- Mate:337: BoardNew2-CZ:7 ↔ Aluminium:18
- Mate:338: Boardborder:1 ↔ Aluminium:18
- Mate:339: BoardNew2-CZ:7 ↔ Aluminium:18
## Named parameters: d21_d20 = 0 mm, d22_d4 = 0 mm, d23_d5 = 0 mm, d24_d6 = 0 mm, d25_d7 = 0 mm, d26_d8 = 0 mm, d27_d9 = 0 mm, d28_d10 = 0 mm, d29_d11 = 0 mm, d66_d20 = 0 mm, d79_d4 = 0 mm, d80_d5 = 0 mm, d81_d6 = 0 mm, d82_d7 = 0 mm, d83_d8 = 0 mm, d84_d9 = 0 mm, d85_d10 = 0 mm, d86_d11 = 0 mm, d182_d161 = 0 mm, d183_d162 = 0 mm, d184_d163 = 0 mm, d185_d164 = 0 mm, d186_d165 = 0 mm, d187_d166 = 0 mm, d188_d167 = 0 mm, d189_d168 = 0 mm, d190_d169 = 0 mm, d191_d103 = 0 mm, d192_d104 = 0 mm, d193_d105 = 0 mm, d194_d54 = 0 mm, d195_d55 = 0 mm, d196_d56 = 0 mm, d197_d57 = 0 mm, d198_d58 = 0 mm, d199_d59 = 0 mm, d200_d66_d20 = 0 mm, d201_d79_d4 = 0 mm, d202_d80_d5 = 0 mm, d203_d81_d6 = 0 mm, d204_d82_d7 = 0 mm, d205_d83_d8 = 0 mm, d206_d84_d9 = 0 mm, d207_d85_d10 = 0 mm, d208_d86_d11 = 0 mm, d209_d88 = 0 mm, d210_d89 = 0 mm, d211_d90 = 0 mm, d212_d91 = 0 mm, d213_d92 = 0 mm, d214_d93 = 0 mm, d215_d94 = 0 mm, d216_d95 = 0 mm, d217_d96 = 0 mm, d218_d97 = 0 mm, d219_d98 = 0 mm, d220_d99 = 0 mm, d221_d100 = 0 mm, d222_d101 = 0 mm, d223_d102 = 0 mm, d224_d20 = 0 mm, d225_d21_d20 = 0 mm, d226_d22_d4 = 0 mm, d227_d23_d5 = 0 mm, d228_d24_d6 = 0 mm, d229_d25_d7 = 0 mm, d230_d26_d8 = 0 mm, d231_d27_d9 = 0 mm, d232_d28_d10 = 0 mm, d233_d29_d11 = 0 mm, d234_d30 = 0 mm, d235_d31 = 0 mm, d236_d32 = 0 mm, d237_d4 = 0 mm, d238_d5 = 0 mm, d239_d6 = 0 mm, d240_d7 = 0 mm, d241_d8 = 0 mm, d242_d9 = 0 mm, d243_d10 = 0 mm, d244_d11 = 0 mm, d245_d170 = 0 mm, d246_d171 = 0 mm, d247_d172 = 0 mm, d248_d173 = 0 mm, d249_d174 = 0 mm, d250_d175 = 0 mm, d251_d176 = 0 mm, d252_d177 = 0 mm, d253_d178 = 0 mm, d254_d179 = 0 mm, d255_d180 = 0 mm, d256_d181 = 0 mm, d260_d161 = 0 mm, d261_d162 = 0 mm, d262_d163 = 0 mm, d263_d164 = 0 mm, d264_d165 = 0 mm, d265_d166 = 0 mm, d266_d167 = 0 mm, d267_d168 = 0 mm, d268_d169 = 0 mm, d269_d103 = 0 mm, d270_d104 = 0 mm, d271_d105 = 0 mm, d272_d54 = 0 mm, d273_d55 = 0 mm, d274_d56 = 0 mm, d275_d57 = 0 mm, d276_d58 = 0 mm, d277_d59 = 0 mm, d278_d66_d20 = 0 mm, d279_d79_d4 = 0 mm, d280_d80_d5 = 0 mm, d281_d81_d6 = 0 mm, d282_d82_d7 = 0 mm, d283_d83_d8 = 0 mm, d284_d84_d9 = 0 mm, d285_d85_d10 = 0 mm, d286_d86_d11 = 0 mm, d287_d88 = 0 mm, d288_d89 = 0 mm, d289_d90 = 0 mm, d290_d91 = 0 mm, d291_d92 = 0 mm, d292_d93 = 0 mm, d293_d94 = 0 mm, d294_d95 = 0 mm, d295_d96 = 0 mm, d296_d97 = 0 mm, d297_d98 = 0 mm, d298_d99 = 0 mm, d299_d100 = 0 mm, d300_d101 = 0 mm, d301_d102 = 0 mm, d302_d20 = 0 mm, d303_d21_d20 = 0 mm, d304_d22_d4 = 0 mm, d305_d23_d5 = 0 mm, d306_d24_d6 = 0 mm, d307_d25_d7 = 0 mm, d308_d26_d8 = 0 mm, d309_d27_d9 = 0 mm, d310_d28_d10 = 0 mm, d311_d29_d11 = 0 mm, d312_d30 = 0 mm, d313_d31 = 0 mm, d314_d32 = 0 mm, d315_d4 = 0 mm, d316_d5 = 0 mm, d317_d6 = 0 mm, d318_d7 = 0 mm, d319_d8 = 0 mm, d320_d9 = 0 mm, d321_d10 = 0 mm, d322_d11 = 0 mm, d323_d170 = 0 mm, d324_d171 = 0 mm, d325_d172 = 0 mm, d326_d173 = 0 mm, d327_d174 = 0 mm, d328_d175 = 0 mm, d329_d176 = 0 mm, d330_d177 = 0 mm, d331_d178 = 0 mm, d332_d179 = 0 mm, d333_d180 = 0 mm, d334_d181 = 0 mm
